# Autodesk Inventor assembly: motherboard_asm
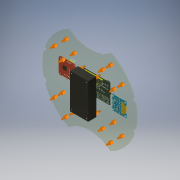
[picture p0: Inventor's stored thumbnail of the model, 180x180]
Saved by Autodesk Inventor 2020 (Build 240168000, 168)
## iProperties
Created: 2024-11-03
Part Number: motherboard_asm
Document SubType Name: Assembly
Designer: Ivan
Mass: 510.508 g
Surface Area: 858.198 cm^2
Volume: 101.338 cm^3
Density: 5.03767 g/cm^3
Author: Ivan
## Documents named in this file (10)
- C:\!projects\DASH-\3D\Dash-V1\motherboard\motherboard_asm.iam
- C:\!projects\DASH-\3D\Dash-V1\motherboard\motherboard.ipt
- C:\!projects\DASH-\3D\Dash-V1\boost.ipt
- C:\!projects\DASH-\3D\Dash-V1\step\m3_bolt\m3x8\Spacer Bolts_m3_bn_L5.ipt
- C:\!projects\DASH-\3D\Dash-V1\step\m3_bolt\Spacer Bolts_m3_bn_L5_ЗЕРКАЛО.ipt
- C:\!projects\DASH-\3D\Dash-V1\step\m3_bolt\Spacer Bolts_m3_bn_L5_ЗЕРКАЛО1.ipt
- C:\!projects\DASH-\3D\Dash-V1\step\m3_bolt\Spacer Bolts_m3_bn_L5_ЗЕРКАЛО_ЗЕРКАЛО.ipt
- C:\!projects\DASH-\3D\Dash-V1\step\mega\MEGA 2560 PRO (EMBED).iam
- C:\!projects\DASH-\3D\Dash-V1\step\SparkFun_9DoF_Razor_IMU\SparkFun 9DoF Razor IMU.ipt
- C:\!projects\DASH-\3D\Dash-V1\step\oled_0.96\Weewooday I2C OLED 0.96'' 128x64.iam
## Components (25 placed, 9 different names)
1. motherboard:1 — Совмещение:1, Совмещение:2, Угол:1, Вставка:1, Вставка:3, Вставка:4, Вставка:6, Вставка:7, Вставка:8, Вставка:9, Вставка:10, Вставка:11, Вставка:12, Вставка:13, Вставка:14, Вставка:15, Вставка:16
2. MEGA 2560 PRO (EMBED):1 [sub-assembly] — Вставка:11, Вставка:12
3. SparkFun 9DoF Razor IMU:1 — Вставка:13, Вставка:14
4. Weewooday I2C OLED 0.96'' 128x64:1 [sub-assembly] — Вставка:15, Вставка:16
5. Spacer Bolts_m3_bn_L5:4 — Вставка:4, Вставка:5
6. Spacer Bolts_m3_bn_L5:3 — Вставка:6
7. Spacer Bolts_m3_bn_L5:2 — Вставка:1
8. Spacer Bolts_m3_bn_L5:1 — Вставка:3, Совмещение:3
9. boost:1 — Вставка:5, Совмещение:3
10. Spacer Bolts_m3_bn_L5:6 — Вставка:8
11. Spacer Bolts_m3_bn_L5:7 — Вставка:7
12. Spacer Bolts_m3_bn_L5:8 — Вставка:10
13. Spacer Bolts_m3_bn_L5_ЗЕРКАЛО:1
14. Spacer Bolts_m3_bn_L5_ЗЕРКАЛО:2
15. Spacer Bolts_m3_bn_L5_ЗЕРКАЛО:3
16. Spacer Bolts_m3_bn_L5_ЗЕРКАЛО:4
17. Spacer Bolts_m3_bn_L5_ЗЕРКАЛО1:1
18. Spacer Bolts_m3_bn_L5_ЗЕРКАЛО1:2
19. Spacer Bolts_m3_bn_L5_ЗЕРКАЛО1:3
20. Spacer Bolts_m3_bn_L5_ЗЕРКАЛО1:4
21. Spacer Bolts_m3_bn_L5_ЗЕРКАЛО_ЗЕРКАЛО:1
22. Spacer Bolts_m3_bn_L5_ЗЕРКАЛО_ЗЕРКАЛО:2
23. Spacer Bolts_m3_bn_L5_ЗЕРКАЛО_ЗЕРКАЛО:3
24. Spacer Bolts_m3_bn_L5_ЗЕРКАЛО_ЗЕРКАЛО:4
25. Spacer Bolts_m3_bn_L5:5 — Вставка:9
## Relationships (19: Insert 15, Mate 3, Angle 1)
- Совмещение:1 [Mate]: motherboard:1
- Совмещение:2 [Mate]: motherboard:1
- Угол:1 [Angle] (-45 deg): motherboard:1
- Вставка:1 [Insert]: motherboard:1 ↔ Spacer Bolts_m3_bn_L5:2
- Вставка:3 [Insert]: motherboard:1 ↔ Spacer Bolts_m3_bn_L5:1
- Вставка:4 [Insert]: motherboard:1 ↔ Spacer Bolts_m3_bn_L5:4
- Вставка:5 [Insert]: Spacer Bolts_m3_bn_L5:4 ↔ boost:1
- Совмещение:3 [Mate]: Spacer Bolts_m3_bn_L5:1 ↔ boost:1
- Вставка:6 [Insert]: motherboard:1 ↔ Spacer Bolts_m3_bn_L5:3
- Вставка:7 [Insert] (5 mm): motherboard:1 ↔ Spacer Bolts_m3_bn_L5:7
- Вставка:8 [Insert] (5 mm): motherboard:1 ↔ Spacer Bolts_m3_bn_L5:6
- Вставка:9 [Insert] (5 mm): motherboard:1 ↔ Spacer Bolts_m3_bn_L5:5
- Вставка:10 [Insert] (5 mm): motherboard:1 ↔ Spacer Bolts_m3_bn_L5:8
- Вставка:11 [Insert] (11 mm): motherboard:1 ↔ MEGA 2560 PRO (EMBED):1
- Вставка:12 [Insert] (11 mm): motherboard:1 ↔ MEGA 2560 PRO (EMBED):1
- Вставка:13 [Insert] (11 mm): motherboard:1 ↔ SparkFun 9DoF Razor IMU:1
- Вставка:14 [Insert] (11 mm): motherboard:1 ↔ SparkFun 9DoF Razor IMU:1
- Вставка:15 [Insert]: motherboard:1 ↔ Weewooday I2C OLED 0.96'' 128x64:1
- Вставка:16 [Insert]: motherboard:1 ↔ Weewooday I2C OLED 0.96'' 128x64:1
